# Autodesk Inventor assembly: project assembly
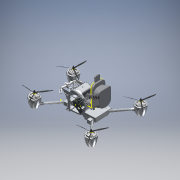
[picture p0: Inventor's stored thumbnail of the model, 180x180]
Saved by Autodesk Inventor 2018 (Build 220112000, 112)
## iProperties
Created: 2021-03-16
Part Number: project assembly
Document SubType Name: Assembly
Designer: abhir
Author: abhir
## Documents named in this file (17)
- C:\Users\Hp\OneDrive\Documents\project assembly.iam
- C:\Users\Hp\OneDrive\Documents\20110002_handlebar.ipt
- C:\Users\Hp\OneDrive\Documents\Front connector.ipt
- C:\Users\Hp\OneDrive\Documents\Main frame.ipt
- C:\Users\Hp\OneDrive\Documents\Rear Connector.ipt
- C:\Users\Hp\OneDrive\Documents\Side frame.ipt
- C:\Users\Hp\OneDrive\Documents\Side frame_MIR1.ipt
- C:\Users\Hp\OneDrive\Documents\arm 5,6.ipt
- C:\Users\Hp\OneDrive\Documents\arm_cup 5,6.ipt
- C:\Users\Hp\OneDrive\Documents\JETENGINE.ipt
- C:\Users\Hp\OneDrive\Documents\arm 5,6_MIR.ipt
- C:\Users\Hp\OneDrive\Documents\arm_cup 5,6_MIR.ipt
- C:\Users\Hp\OneDrive\Documents\JETENGINE_MIR.ipt
- C:\Users\Hp\OneDrive\Documents\final engine.ipt
- C:\Users\Hp\OneDrive\Documents\propeller.ipt
- C:\Users\Hp\OneDrive\Documents\seat suspension final.ipt
- C:\Users\Hp\OneDrive\Documents\seat_final.ipt
## Components (25 placed, 16 different names)
1. Front connector:1 — Mate:1, Transitional:1, Mate:3, Mate:6, Mate:11
2. Main frame:1 — Mate:1, Transitional:1, Mate:2, Rotational:1, Mate:3, Mate:4, Rotational:2, Rotational:3, Angle:1, Mate:16, Mate:17
3. Rear Connector:1 — Mate:2, Rotational:1, Mate:5, Rigid:1
4. 20110002_handlebar:1 — Mate:4
5. side frame:1 — Rotational:2, Rotational:3
6. arm 5,6:1 — Mate:5, Mate:7
7. arm 5,6:2 — Mate:6, Mate:8
8. arm_cup 5,6:1 — Mate:7, Mate:10
9. arm_cup 5,6:2 — Mate:8, Mate:9
10. JETENGINE:1 — Mate:9, Rotational:9
11. JETENGINE:2 — Mate:10, Rotational:8
12. Side frame_MIR1:2
13. arm 5,6_MIR:1 — Mate:12
14. arm 5,6_MIR:2 — Mate:13
15. arm_cup 5,6_MIR:1 — Mate:12, Mate:15
16. arm_cup 5,6_MIR:2 — Mate:13, Mate:14
17. JETENGINE_MIR:1 — Mate:14, Rotational:10
18. JETENGINE_MIR:2 — Mate:15, Rotational:11
19. final engine:1 — Mate:16, Mate:17
20. propeller:1 — Rotational:8
21. propeller:2 — Rotational:11
22. propeller:3 — Rotational:9
23. propeller:4 — Rotational:10
24. seat suspension final:1 — Rigid:1, Mate:18, Mate:19
25. seat_final:1 — Mate:18, Mate:19
## Relationships (29: Mate 19, RevoluteJoint 7, Transitional 1, Angle 1, WeldJoint 1)
- Mate:1: Front connector:1 ↔ Main frame:1
- Transitional:1: Front connector:1 ↔ Main frame:1
- Mate:2: Main frame:1 ↔ Rear Connector:1
- Rotational:1 [RevoluteJoint]: Main frame:1 ↔ Rear Connector:1
- Mate:3: Front connector:1 ↔ Main frame:1
- Mate:4: Main frame:1 ↔ 20110002_handlebar:1
- Rotational:2 [RevoluteJoint]: Main frame:1 ↔ side frame:1
- Rotational:3 [RevoluteJoint]: Main frame:1 ↔ side frame:1
- Mate:5: Rear Connector:1 ↔ arm 5,6:1
- Mate:6: Front connector:1 ↔ arm 5,6:2
- Mate:7: arm 5,6:1 ↔ arm_cup 5,6:1
- Mate:8: arm 5,6:2 ↔ arm_cup 5,6:2
- Mate:9: arm_cup 5,6:2 ↔ JETENGINE:1
- Mate:10: arm_cup 5,6:1 ↔ JETENGINE:2
- Mate:11: Front connector:1
- Angle:1 (0 deg): Main frame:1
- Mate:12: arm 5,6_MIR:1 ↔ arm_cup 5,6_MIR:1
- Mate:13: arm 5,6_MIR:2 ↔ arm_cup 5,6_MIR:2
- Mate:14: arm_cup 5,6_MIR:2 ↔ JETENGINE_MIR:1
- Mate:15: arm_cup 5,6_MIR:1 ↔ JETENGINE_MIR:2
- Mate:16: Main frame:1 ↔ final engine:1
- Mate:17: Main frame:1 ↔ final engine:1
- Rotational:8 [RevoluteJoint]: JETENGINE:2 ↔ propeller:1
- Rigid:1 [WeldJoint]: Rear Connector:1 ↔ seat suspension final:1
- Rotational:9 [RevoluteJoint]: JETENGINE:1 ↔ propeller:3
- Rotational:10 [RevoluteJoint]: JETENGINE_MIR:1 ↔ propeller:4
- Rotational:11 [RevoluteJoint]: JETENGINE_MIR:2 ↔ propeller:2
- Mate:18: seat suspension final:1 ↔ seat_final:1
- Mate:19: seat suspension final:1 ↔ seat_final:1
